# Autodesk Inventor assembly: Belt Tensioner End
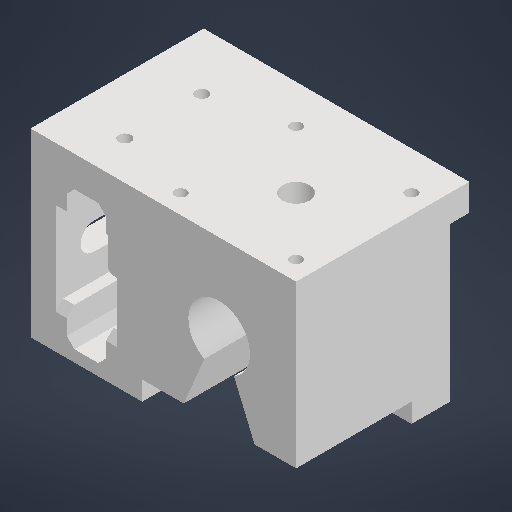
[picture p0: Inventor's stored thumbnail of the model, 512x512]
Saved by Autodesk Inventor 2025.1 (Build 291241000, 241)
## iProperties
Created: 2025-02-02
Part Number: Belt Tensioner End
Document SubType Name: Assembly
Designer: jerem
Author: jerem
## Documents named in this file (7)
- C:\Users\jerem\Documents\GitHub\Perovskite-Automated-Synthesis-System\CAD\Gantry\Belt Tensioner End.iam
- C:\Users\jerem\Documents\GitHub\Perovskite-Automated-Synthesis-System\CAD\Gantry\Idlert Tensioner.ipt
- C:\Users\jerem\Documents\GitHub\Perovskite-Automated-Synthesis-System\CAD\Gantry\tensionerholder.ipt
- C:\Users\jerem\Documents\GitHub\Perovskite-Automated-Synthesis-System\CAD\Gantry\X Axis End.ipt
- C:\Users\jerem\Documents\GitHub\Perovskite-Automated-Synthesis-System\CAD\Gantry\Tensioner Top.ipt
- C:\Users\jerem\Documents\GitHub\Perovskite-Automated-Synthesis-System\CAD\Non 3D Printed Parts\Screws\M3x12.ipt
- C:\Users\jerem\Documents\GitHub\Perovskite-Automated-Synthesis-System\CAD\Gantry\screwer.ipt
## Components (6 placed, 6 different names)
1. Idlert Tensioner:1 — Angle:1, Angle:2, Mate:8, Mate:9, Mate:10
2. tensionerholder:1 — Flush:1, Flush:2, Mate:1, Angle:1, Angle:2, Mate:8, Mate:14
3. X Axis End:1 — Flush:1, Flush:2, Mate:1, Mate:5, Mate:6, Mate:7
4. Tensioner Top:1 — Mate:5, Mate:6, Mate:7
5. M3x12:1 — Mate:9, Mate:10, Rotation/Translation:1, Mate:15
6. screwer:1 — Mate:14, Rotation/Translation:1, Mate:15
## Relationships (14: Mate 9, Flush 2, Angle 2, RelateRotateTranslate 1)
- Flush:1: tensionerholder:1 ↔ X Axis End:1
- Flush:2: tensionerholder:1 ↔ X Axis End:1
- Mate:1: tensionerholder:1 ↔ X Axis End:1
- Angle:1 (180 deg): Idlert Tensioner:1 ↔ tensionerholder:1
- Angle:2 (0 deg): Idlert Tensioner:1 ↔ tensionerholder:1
- Mate:5: X Axis End:1 ↔ Tensioner Top:1
- Mate:6: X Axis End:1 ↔ Tensioner Top:1
- Mate:7: X Axis End:1 ↔ Tensioner Top:1
- Mate:8: Idlert Tensioner:1 ↔ tensionerholder:1
- Mate:9: Idlert Tensioner:1 ↔ M3x12:1
- Mate:10: Idlert Tensioner:1 ↔ M3x12:1
- Mate:14: tensionerholder:1 ↔ screwer:1
- Rotation/Translation:1 [RelateRotateTranslate] (1 mm): M3x12:1 ↔ screwer:1
- Mate:15: M3x12:1 ↔ screwer:1
